# Autodesk Inventor assembly: assembly
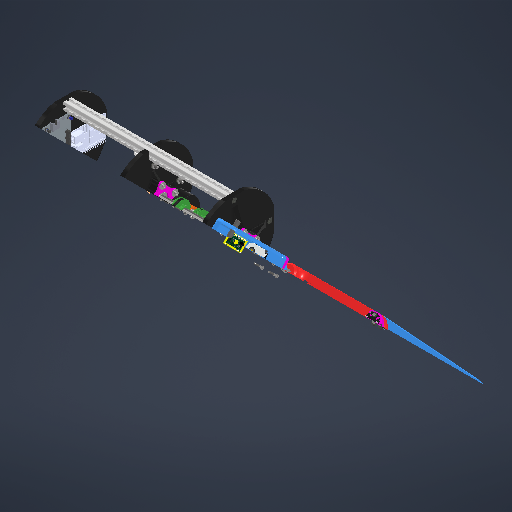
[picture p0: Inventor's stored thumbnail of the model, 512x512]
Saved by Autodesk Inventor 2027.1 (Build 311270010, 270A)
## iProperties
Created: 2026-10-07
Part Number: assembly
Document SubType Name: Assembly
Designer: luca
Author: luca
## Documents named in this file (71)
- C:\Users\lucao\Desktop\RL-Rotary-Inverted-Double-Pendulum\CAD\assembly.iam
- C:\Users\lucao\Desktop\RL-Rotary-Inverted-Double-Pendulum\CAD\motor\L-7015-251029\2D3D\RMD-7015三维图\RMD-7015\RMD-7015.ipt
- C:\Users\lucao\Desktop\RL-Rotary-Inverted-Double-Pendulum\CAD\encoder\AMT102-D2048-I6350-S\3D\AMT102-D2048-I6350-S\AMT102-D2048-I6350-S.ipt
- C:\Users\lucao\Desktop\RL-Rotary-Inverted-Double-Pendulum\CAD\Electronics\RASPBERRY_PI_5\RASPBERRY_PI_5.ipt
- C:\Users\lucao\Desktop\RL-Rotary-Inverted-Double-Pendulum\CAD\Electronics\stm32\NUCLEO-F429ZI--3DModel-STEP-56544\NUCLEO-F429ZI--3DModel-STEP-56544.ipt
- C:\Users\lucao\Desktop\RL-Rotary-Inverted-Double-Pendulum\CAD\al-profil-20x20-drazka-6\al-profil-20x20-drazka-6.ipt
- C:\Users\lucao\Desktop\RL-Rotary-Inverted-Double-Pendulum\CAD\plate_lower.ipt
- C:\Users\lucao\Desktop\RL-Rotary-Inverted-Double-Pendulum\CAD\plate_middle.ipt
- C:\Users\lucao\Desktop\RL-Rotary-Inverted-Double-Pendulum\CAD\drive_shaft_center.ipt
- C:\Users\lucao\Desktop\RL-Rotary-Inverted-Double-Pendulum\CAD\plate_upper.ipt
- C:\Users\lucao\Desktop\RL-Rotary-Inverted-Double-Pendulum\CAD\motor_driveshaft.ipt
- C:\Users\lucao\Desktop\RL-Rotary-Inverted-Double-Pendulum\CAD\90_Deg_Profile\90_Deg_Profile.ipt
- C:\Users\lucao\Desktop\RL-Rotary-Inverted-Double-Pendulum\CAD\pulleyGT3_12mm.ipt
- C:\Users\lucao\Desktop\RL-Rotary-Inverted-Double-Pendulum\CAD\pulleyGT3_17mm.ipt
- C:\Users\lucao\Documents\Inventor\Content Center Files\R2027\en-US\DIN 625 - T1\DIN 625 T1 - 16003 - 17 x 35 x 8.ipt
- C:\Users\lucao\Desktop\RL-Rotary-Inverted-Double-Pendulum\CAD\motor_flange.ipt
- C:\Users\lucao\Documents\Inventor\Content Center Files\R2027\en-US\DIN EN ISO 7091\DIN EN ISO 7091 - 4.ipt
- C:\Users\lucao\Documents\Inventor\Content Center Files\R2027\en-US\ISO 4762(1)\DIN EN ISO 4762 - M4 x 20.ipt
- C:\Users\lucao\Documents\Inventor\Content Center Files\R2027\en-US\ISO 4032(1)\ISO 4032 - M4DIN EN.ipt
- C:\Users\lucao\Documents\Inventor\Content Center Files\R2027\en-US\DIN 914\DIN 914 - M4 x 12.ipt
- C:\Users\lucao\Desktop\RL-Rotary-Inverted-Double-Pendulum\CAD\bearing_lock_middleplate_upper.ipt
- C:\Users\lucao\Desktop\RL-Rotary-Inverted-Double-Pendulum\CAD\bearing_distancer_middle.ipt
- C:\Users\lucao\Documents\Inventor\Content Center Files\R2027\en-US\DIN 9021\DIN 9021 - 5,3.ipt
- C:\Users\lucao\Documents\Inventor\Content Center Files\R2027\en-US\ISO 4762(1)\DIN EN ISO 4762 - M5 x 40.ipt
- C:\Users\lucao\Documents\Inventor\Content Center Files\R2027\en-US\ISO 4032(1)\ISO 4032 - M5DIN EN.ipt
- C:\Users\lucao\Documents\Inventor\Content Center Files\R2027\en-US\ISO 4762(1)\DIN EN ISO 4762 - M3 x 16.ipt
- C:\Users\lucao\Documents\Inventor\Content Center Files\R2027\en-US\DIN EN ISO 7091\DIN EN ISO 7091 - 3.ipt
- C:\Users\lucao\Desktop\RL-Rotary-Inverted-Double-Pendulum\CAD\timing_belt.ipt
- C:\Users\lucao\Documents\Inventor\Content Center Files\R2027\en-US\ISO 10642(2)\ISO 10642  - M6  x  45.ipt
- C:\Users\lucao\Documents\Inventor\Content Center Files\R2027\en-US\ISO 4762(1)\DIN EN ISO 4762 - M6 x 25.ipt
- C:\Users\lucao\Documents\Inventor\Content Center Files\R2027\en-US\ISO 7091\ISO 7091 - ST 6 - 100 HV.ipt
- C:\Users\lucao\Documents\Inventor\Content Center Files\R2027\en-US\ISO 4036(1)\ISO 4036 - M6(1).ipt
- C:\Users\lucao\Desktop\RL-Rotary-Inverted-Double-Pendulum\CAD\axialLock_mainShaft.ipt
- C:\Users\lucao\Documents\Inventor\Content Center Files\R2027\en-US\DIN 914\DIN 914 - M3 x 6.ipt
- C:\Users\lucao\Documents\Inventor\Content Center Files\R2027\en-US\DIN EN ISO 4036\DIN EN ISO 4036 - M3.ipt
- C:\Users\lucao\Desktop\RL-Rotary-Inverted-Double-Pendulum\CAD\link_mainaxis_to_horArm.ipt
- C:\Users\lucao\Documents\Inventor\Content Center Files\R2027\en-US\DIN BEARING(1)\DIN 625 SKF - SKF 6001.ipt
- C:\Users\lucao\Desktop\RL-Rotary-Inverted-Double-Pendulum\CAD\drive_shaft_arm.ipt
- C:\Users\lucao\Desktop\RL-Rotary-Inverted-Double-Pendulum\CAD\slipringMountArm.ipt
- C:\Users\lucao\Desktop\RL-Rotary-Inverted-Double-Pendulum\CAD\slipRing.ipt
- C:\Users\lucao\Desktop\RL-Rotary-Inverted-Double-Pendulum\CAD\distanceTube_armshaft.ipt
- C:\Users\lucao\Desktop\RL-Rotary-Inverted-Double-Pendulum\CAD\slipRingMount_mainAxis.ipt
- C:\Users\lucao\Desktop\RL-Rotary-Inverted-Double-Pendulum\CAD\plate_arm_bearing_fix.ipt
- C:\Users\lucao\Documents\Inventor\Content Center Files\R2027\en-US\DIN 6912\DIN 6912 - M4 x 25.ipt
- C:\Users\lucao\Desktop\RL-Rotary-Inverted-Double-Pendulum\CAD\slipring_tube.ipt
- C:\Users\lucao\Desktop\RL-Rotary-Inverted-Double-Pendulum\CAD\Insert M3 D5 L5mm\Insert M3 D5 L5mm.ipt
- C:\Users\lucao\Documents\Inventor\Content Center Files\R2027\en-US\CNS 4481\CNS 4481 - M3 x 5.ipt
- C:\Users\lucao\Documents\Inventor\Content Center Files\R2027\en-US\CNS 4481\CNS 4481 - M3 x 6.ipt
- C:\Users\lucao\Documents\Inventor\Content Center Files\R2027\en-US\DIN 7984\DIN 7984 - M3 x 6.ipt
- C:\Users\lucao\Desktop\RL-Rotary-Inverted-Double-Pendulum\CAD\STM32 Mini F401\STM32MiniF401.iam
- C:\Users\lucao\Desktop\RL-Rotary-Inverted-Double-Pendulum\CAD\weight_rod.ipt
- C:\Users\lucao\Desktop\RL-Rotary-Inverted-Double-Pendulum\CAD\axialLock_arm.ipt
- C:\Users\lucao\Documents\Inventor\Content Center Files\R2027\en-US\DIN 914\DIN 914 - M3 x 8.ipt
- C:\Users\lucao\Desktop\RL-Rotary-Inverted-Double-Pendulum\CAD\pendulum_1.ipt
- C:\Users\lucao\Documents\Inventor\Content Center Files\R2027\en-US\DIN BEARING(1)\DIN 625 SKF - SKF 608.ipt
- C:\Users\lucao\Desktop\RL-Rotary-Inverted-Double-Pendulum\CAD\pendulum_2.ipt
- C:\Users\lucao\Desktop\RL-Rotary-Inverted-Double-Pendulum\CAD\rod_link1to2.ipt
- C:\Users\lucao\Documents\Inventor\Content Center Files\R2027\en-US\DIN 7349\DIN 7349 - 4,3.ipt
- C:\Users\lucao\Documents\Inventor\Content Center Files\R2027\en-US\CSN EN 24017\ISO 4017 - M4 x 8CSN EN.ipt
- C:\Users\lucao\Desktop\RL-Rotary-Inverted-Double-Pendulum\CAD\sensormout_pendulum.ipt
- C:\Users\lucao\Desktop\RL-Rotary-Inverted-Double-Pendulum\CAD\mt6701.ipt
- C:\Users\lucao\Desktop\RL-Rotary-Inverted-Double-Pendulum\CAD\magnet.ipt
- C:\Users\lucao\Desktop\RL-Rotary-Inverted-Double-Pendulum\CAD\Insert M3 D5 L5mm\Insert M3 D5 L5mm_MIR.ipt
- C:\Users\lucao\Documents\Inventor\Content Center Files\R2027\en-US\DIN 7349\DIN 7349 - 3,2.ipt
- C:\Users\lucao\Documents\Inventor\Content Center Files\R2027\en-US\ISO 4762(1)\DIN EN ISO 4762 - M3 x 8.ipt
- C:\Users\lucao\Documents\Inventor\Content Center Files\R2027\en-US\ISO 10642(2)\ISO 10642  - M3  x  16.ipt
- C:\Users\lucao\Documents\Inventor\Content Center Files\R2027\en-US\DIN EN 24 036(2)\DIN EN 24 036 - M3.ipt
- C:\Users\lucao\Desktop\RL-Rotary-Inverted-Double-Pendulum\CAD\Insert M3 D5 L5mm\Insert M3 D5 L5mm_MIR1.ipt
- C:\Users\lucao\Documents\Inventor\Content Center Files\R2027\en-US\ISO 10642(2)\ISO 10642  - M3  x  10.ipt
- C:\Users\lucao\Documents\Inventor\Content Center Files\R2027\en-US\DIN EN ISO 4027\DIN EN ISO 4027 - M3 x 16.ipt
- C:\Users\lucao\Desktop\RL-Rotary-Inverted-Double-Pendulum\CAD\Insert M3 D5 L5mm\Insert M3 D5 L5mm_MIR2.ipt
## Components (197 placed, 70 different names)
1. RASPBERRY_PI_5:1 — Mate:7
2. NUCLEO-F429ZI--3DModel-STEP-56544:1 — Mate:6
3. timing_belt:1 — Mate:91, Mate:92, Mate:93
4. RMD-7015:1 — Mate:11, Mate:34, Mate:35, Angle:4, Mate:57, Mate:58, Mate:72, Mate:74, Mate:75, Mate:76, Mate:77, Mate:78
5. motor_driveshaft:1 — Mate:34, Mate:35, Mate:55, Mate:56, Mate:91
6. pulleyGT3_12mm:1 — Mate:55, Mate:71, Flush:5, Mate:93
7. motor_flange:1 — Mate:56, Mate:57, Insert:1, Insert:2, Insert:3, Insert:4, Insert:9, Mate:58, Flush:4, Mate:71
8. DIN EN ISO 7091 4:1 — Insert:1, Insert:5
9. DIN EN ISO 7091 4:2 — Insert:2, Insert:8
10. DIN EN ISO 7091 4:3 — Insert:3, Insert:7
11. DIN EN ISO 7091 4:4 — Insert:4, Insert:6
12. DIN EN ISO 4762 M4 x 20:1 — Insert:5
13. DIN EN ISO 4762 M4 x 20:2 — Insert:6
14. DIN EN ISO 4762 M4 x 20:3 — Insert:7
15. DIN EN ISO 4762 M4 x 20:4 — Insert:8
16. DIN 625 - T1 16003 - 17 x 35 x 8:4 — Mate:53, Mate:132, Mate:133, Mate:136
17. DIN 625 - T1 16003 - 17 x 35 x 8:3 — Mate:52, Mate:129, Mate:131, Mate:149
18. DIN 625 - T1 16003 - 17 x 35 x 8:2 — Mate:51, Mate:63, Mate:69
19. DIN 625 - T1 16003 - 17 x 35 x 8:1 — Mate:50, Mate:65, Mate:67, Mate:70, Flush:6
20. DIN EN 24032 M5:4 — Insert:22
21. DIN EN 24032 M5:3 — Insert:21
22. DIN EN 24032 M5:2 — Insert:20
23. DIN EN 24032 M5:1 — Insert:19
24. DIN EN ISO 7091 3:4 — Mate:85, Mate:86, Mate:90
25. DIN EN ISO 7091 3:3 — Mate:83, Mate:84, Mate:89
26. DIN EN ISO 7091 3:2 — Mate:81, Mate:82, Mate:87
27. DIN EN ISO 7091 3:1 — Mate:79, Mate:80, Mate:88
28. DIN EN ISO 4762 M3 x 16:4 — Mate:77, Mate:79, Mate:88
29. DIN EN ISO 4762 M3 x 16:3 — Mate:76, Mate:83, Mate:89
30. DIN EN ISO 4762 M3 x 16:2 — Mate:78, Mate:85, Mate:90
31. DIN EN ISO 4762 M3 x 16:1 — Mate:75, Mate:81, Mate:87
32. bearing_distancer_middle:2 — Mate:130, Mate:131, Mate:132
33. bearing_distancer_middle:1 — Mate:68, Mate:69, Mate:70
34. plate_lower:1 — Mate:1, Mate:2, Mate:3, Mate:4, Mate:5, Angle:1, Mate:6, Mate:7, Mate:17, Mate:19, Mate:98, Mate:99, Mate:100, Mate:101
35. DIN EN ISO 10642 M6  x  45:4 — Mate:97
36. DIN EN ISO 10642 M6  x  45:2 — Mate:95
37. DIN EN ISO 10642 M6  x  45:1 — Mate:94
38. DIN EN ISO 10642 M6  x  45:3 — Mate:96
39. DIN EN ISO 10642 M6  x  45:6 — Mate:99
40. DIN EN ISO 10642 M6  x  45:7 — Mate:100
41. DIN EN ISO 10642 M6  x  45:5 — Mate:98
42. DIN EN ISO 10642 M6  x  45:8 — Mate:101
43. plate_middle:1 — Mate:11, Mate:17, Mate:19, Angle:2, Mate:42, Mate:62, Mate:66, Mate:67, Insert:14, Mate:80, Mate:82, Mate:84, Mate:86, Mate:102, Mate:104, Mate:106, Mate:108, Mate:111, Mate:113, Mate:115, Mate:117
44. plate_upper:1 — Mate:18, Mate:20, Mate:21, Angle:3, Mate:94, Mate:95, Mate:96, Mate:97, Mate:133, Mate:134, Mate:142
45. bearing_lock_middleplate_upper:1 — Mate:61, Mate:62, Mate:63, Insert:10, Insert:11, Insert:12, Insert:13
46. DIN 9021 5,3:1 — Insert:10, Insert:18
47. DIN 9021 5,3:2 — Insert:11, Insert:17
48. DIN 9021 5,3:3 — Insert:12, Insert:15
49. DIN 9021 5,3:4 — Insert:13, Insert:16
50. DIN EN ISO 4762 M5 x 40:1 — Insert:15
51. DIN EN ISO 4762 M5 x 40:2 — Insert:16
52. DIN EN ISO 4762 M5 x 40:3 — Insert:17
53. DIN EN ISO 4762 M5 x 40:4 — Insert:18
54. DIN EN ISO 4762 M6 x 25:1 — Mate:102, Mate:103, Mate:110, Mate:120
55. DIN EN ISO 4762 M6 x 25:2 — Mate:104, Mate:105, Mate:116, Mate:118
56. DIN EN ISO 4762 M6 x 25:3 — Mate:106, Mate:107, Mate:114, Mate:122
57. DIN EN ISO 4762 M6 x 25:4 — Mate:108, Mate:109, Mate:112, Mate:124
58. ISO 7091 ST 6 - 100 HV:1 — Mate:110, Mate:111, Mate:121
59. ISO 7091 ST 6 - 100 HV:2 — Mate:112, Mate:113, Mate:125
60. ISO 7091 ST 6 - 100 HV:3 — Mate:114, Mate:115, Mate:123
61. ISO 7091 ST 6 - 100 HV:4 — Mate:116, Mate:117, Mate:119
62. DIN EN 24036 M6:1 — Mate:118, Mate:119
63. DIN EN 24036 M6:2 — Mate:120, Mate:121
64. DIN EN 24036 M6:3 — Mate:122, Mate:123
65. DIN EN 24036 M6:4 — Mate:124, Mate:125
66. bearing_lock_middleplate_upper:2 — Mate:128, Mate:129, Mate:134, Mate:137, Mate:139
67. axialLock_arm:1 — Mate:194, Mate:195, Mate:196, Angle:9, Mate:197, Mate:198, Mate:199
68. slipRing:1 — Mate:178, Flush:9
69. slipring_tube:1 — Mate:176, Mate:177, Mate:178, Flush:9, Flush:13
70. slipringMountArm:1 — Mate:174, Mate:175, Mate:179, Flush:10, Mate:180, Flush:11, Mate:181, Mate:182, Mate:183, Flush:12
71. drive_shaft_arm:1 — Mate:154, Mate:158, Mate:165, Flush:8, Mate:174, Mate:176, Mate:194, Mate:202, Flush:17
72. pendulum_1:1 — Mate:202, Flush:17, Mate:203, Mate:217, Mate:219, Mate:223, Mate:234, Angle:11, Mate:235, Flush:20, Mate:240, Mate:241, Angle:12, Flush:22, Flush:23, Mate:249, Flush:29
73. DIN 625 SKF SKF 608:1 — Mate:203, Mate:206, Mate:208, Mate:211, Mate:220, Mate:223
74. sensormout_pendulum:1 — Mate:217, Mate:219, Mate:220, Mate:222, Mate:229, Flush:19, Mate:232, Mate:236, Mate:237, Flush:21, Mate:248
75. mt6701:1 — Mate:221, Mate:222, Mate:226, Mate:230, Mate:231, Mate:239
76. Insert M3 D5 L5mm:11 — Mate:229, Flush:19
77. Insert M3 D5 L5mm_MIR:1 — Flush:21, Mate:238
78. DIN 7349 3,2:1 — Mate:230, Mate:231, Insert:34
79. DIN EN ISO 4762 M3 x 8:1 — Insert:34
80. DIN 7349 3,2:2 — Insert:35, Mate:239
81. DIN EN ISO 4762 M3 x 8:2 — Insert:35, Mate:238, Mate:248
82. DIN EN ISO 10642 M3  x  16:1 — Mate:232, Mate:233
83. DIN EN 24036 M3:1 — Mate:233, Mate:234, Angle:11
84. Insert M3 D5 L5mm:12 — Mate:235, Flush:20
85. Insert M3 D5 L5mm_MIR1:1 — Mate:249, Flush:29
86. DIN EN ISO 10642 M3  x  10:1 — Mate:236
87. DIN EN ISO 10642 M3  x  10:2 — Mate:237
88. DIN EN 24032 M4:9 — Mate:240, Mate:241, Angle:12, Mate:242
89. DIN 914 M4 x 12:5 — Mate:242, Flush:22
90. AMT102-D2048-I6350-S:1 — Mate:173, Angle:7, Mate:177, Flush:13, Mate:187, Mate:189
91. pulleyGT3_17mm:1 — Mate:54, Flush:5
92. drive_shaft_center:1 — Mate:50, Mate:51, Mate:52, Mate:53, Mate:54, Mate:61, Mate:66, Mate:68, Mate:72, Mate:92, Mate:128, Mate:130, Mate:135, Flush:6, Flush:7, Mate:148, Mate:161, Mate:162, Angle:8
93. DIN 625 SKF SKF 6001:2 — Mate:151, Mate:160, Mate:164, Mate:175
94. DIN 625 SKF SKF 6001:3 — Mate:154, Mate:159, Mate:163, Mate:190, Mate:195
95. distanceTube_armshaft:1 — Mate:158, Mate:159, Mate:160
96. slipRingMount_mainAxis:1 — Mate:161, Mate:162, Mate:243, Flush:24
97. plate_arm_bearing_fix:1 — Mate:165, Mate:166, Insert:25, Insert:26, Insert:27, Insert:28, Mate:190
98. DIN EN ISO 7091 4:7 — Insert:25, Insert:29
99. DIN EN ISO 7091 4:8 — Insert:26, Insert:30
100. DIN EN ISO 7091 4:9 — Insert:27, Insert:31
101. DIN EN ISO 7091 4:10 — Insert:28, Insert:32
102. DIN 6912 M4 x 25:1 — Insert:29, Mate:200
103. DIN 6912 M4 x 25:2 — Insert:30
104. DIN 6912 M4 x 25:3 — Insert:31
105. DIN 6912 M4 x 25:4 — Insert:32
106. Insert M3 D5 L5mm:9 — Mate:184, Flush:14
107. Insert M3 D5 L5mm:10 — Mate:185, Flush:15
108. DIN 7984 M3 x 6:1 — Mate:186, Mate:187
109. DIN 7984 M3 x 6:2 — Mate:188, Mate:189
110. STM32MiniF401:1 [sub-assembly] — Mate:191, Mate:192
111. weight_rod:1 — Mate:193, Flush:16
112. DIN EN 24032 M4:5 — Mate:200, Mate:201, Angle:10
113. DIN EN 24032 M4:6
114. DIN EN 24032 M4:7
115. DIN EN 24032 M4:8
116. slipRing:2 — Mate:243, Flush:24
117. Insert M3 D5 L5mm:13 — Mate:244, Flush:25, Mate:245
118. DIN EN ISO 4027 M3 x 16:1 — Mate:245, Flush:28
119. Insert M3 D5 L5mm_MIR2:1 — Mate:246, Mate:247, Flush:26
120. DIN EN ISO 4027 M3 x 16:2 — Mate:246, Flush:27
121. axialLock_mainShaft:1 — Mate:135, Mate:136, Mate:145, Angle:6, Mate:147
122. link_mainaxis_to_horArm:1 — Mate:148, Mate:149, Mate:151, Mate:152, Mate:163, Mate:164, Mate:166, Mate:173, Angle:7, Flush:8, Mate:184, Flush:14, Mate:185, Flush:15, Mate:186, Mate:188, Angle:8, Mate:191, Mate:192, Mate:193, Flush:16, Mate:201, Angle:10, Mate:244, Flush:25, Mate:247, Flush:26, Flush:27, Flush:28
123. magnet:1 — Mate:224, Mate:225, Mate:226
124. pendulum_2:1 — Mate:206, Mate:208, Mate:209, Flush:18, Mate:213
125. rod_link1to2:1 — Mate:209, Flush:18, Mate:210, Mate:212, Mate:214
126. DIN 7349 4,3:1 — Mate:210, Mate:211, Insert:33, Mate:221, Mate:225
127. DIN 7349 4,3:2 — Mate:212, Mate:213, Mate:215
128. CSN EN 24017 M4 x 8:1 — Insert:33, Mate:224
129. CSN EN 24017 M4 x 8:2 — Mate:214, Mate:215
130. DIN EN 24032 M4:1 — Insert:9, Mate:59
131. DIN EN 24032 M4:2
132. DIN EN 24032 M4:3
133. DIN EN 24032 M4:4
134. DIN 914 M4 x 12:1 — Mate:59, Flush:4
135. DIN 914 M4 x 12:2
136. DIN 914 M4 x 12:3
137. DIN 914 M4 x 12:4
138. DIN 9021 5,3:5 — Insert:14, Insert:22
139. DIN 9021 5,3:6 — Insert:21
140. DIN 9021 5,3:7 — Insert:20
141. DIN 9021 5,3:8 — Insert:19
142. al-profil-20x20-drazka-6:1 — Mate:4, Mate:5, Angle:1, Mate:20, Mate:21
143. al-profil-20x20-drazka-6:2 — Mate:18, Angle:2, Angle:3
144. al-profil-20x20-drazka-6:3
145. al-profil-20x20-drazka-6:4 — Flush:1, Mate:43
146. 90_Deg_Profile:1 — Mate:42, Flush:1, Mate:43, Mate:103, Mate:105, Mate:107, Mate:109
147. 90_Deg_Profile:2
148. 90_Deg_Profile:3
149. 90_Deg_Profile:4
150. DIN EN 24032 M5:5 — Mate:143, Mate:144
151. DIN EN ISO 4762 M5 x 40:5 — Mate:137, Mate:138, Mate:140, Mate:141, Mate:144
152. DIN 9021 5,3:10 — Mate:141, Mate:142, Mate:143
153. DIN 9021 5,3:9 — Mate:138, Mate:139, Mate:140
154. DIN EN 24032 M5:6
155. DIN EN ISO 4762 M5 x 40:6
156. DIN 9021 5,3:11
157. DIN 9021 5,3:12
158. DIN EN 24032 M5:7
159. DIN EN ISO 4762 M5 x 40:7
160. DIN 9021 5,3:13
161. DIN 9021 5,3:14
162. DIN EN 24032 M5:8
163. DIN EN ISO 4762 M5 x 40:8
164. DIN 9021 5,3:15
165. DIN 9021 5,3:16
166. DIN 914 M3 x 8:1 — Mate:198, Mate:199
167. DIN 914 M3 x 8:2
168. DIN 914 M3 x 8:3
169. DIN 914 M3 x 8:4
170. DIN EN ISO 4036 M3:5 — Mate:196, Angle:9, Mate:197
171. DIN EN ISO 4036 M3:6
172. DIN EN ISO 4036 M3:7
173. DIN EN ISO 4036 M3:8
174. Insert M3 D5 L5mm:1 — Mate:179, Flush:10
175. Insert M3 D5 L5mm:2
176. Insert M3 D5 L5mm:3
177. Insert M3 D5 L5mm:4
178. Insert M3 D5 L5mm:5 — Mate:180, Flush:11
179. Insert M3 D5 L5mm:6
180. Insert M3 D5 L5mm:7
181. Insert M3 D5 L5mm:8
182. CNS 4481 M3 x 5:1 — Mate:181, Mate:182
183. CNS 4481 M3 x 5:2
184. CNS 4481 M3 x 5:3
185. CNS 4481 M3 x 5:4
186. CNS 4481 M3 x 6:3 — Mate:183, Flush:12
187. CNS 4481 M3 x 6:4
188. CNS 4481 M3 x 6:5
189. CNS 4481 M3 x 6:6
190. DIN 914 M3 x 6:1 — Mate:145, Flush:7
191. DIN 914 M3 x 6:2 — Mate:146
192. DIN 914 M3 x 6:3
193. DIN 914 M3 x 6:4
194. DIN EN ISO 4036 M3:1 — Mate:146, Angle:6, Mate:147
195. DIN EN ISO 4036 M3:2
196. DIN EN ISO 4036 M3:3
197. DIN EN ISO 4036 M3:4
## Component patterns: (4 elements, first: DIN EN 24032 M4:1), (4 elements, first: DIN 914 M4 x 12:1), (4 elements, first: DIN 9021 5,3:5), (4 elements, first: al-profil-20x20-drazka-6:1), (4 elements, first: 90_Deg_Profile:1), (4 elements, first: DIN EN 24032 M5:5 + DIN EN ISO 4762 M5 x 40:5 + DIN 9021 5,3:10 + DIN 9021 5,3:9), (4 elements, first: DIN 914 M3 x 8:1), (4 elements, first: DIN EN ISO 4036 M3:5), (4 elements, first: Insert M3 D5 L5mm:1), (4 elements, first: Insert M3 D5 L5mm:5), (4 elements, first: CNS 4481 M3 x 5:1), (4 elements, first: CNS 4481 M3 x 6:3), (4 elements, first: DIN 914 M3 x 6:1), (4 elements, first: DIN EN ISO 4036 M3:1)
## Relationships (267: Mate 195, Insert 33, Flush 27, Angle 12)
- Mate:1: plate_lower:1
- Mate:2: plate_lower:1
- Mate:3: plate_lower:1
- Mate:4: plate_lower:1 ↔ al-profil-20x20-drazka-6:1
- Mate:5: plate_lower:1 ↔ al-profil-20x20-drazka-6:1
- Angle:1 (0 deg): plate_lower:1 ↔ al-profil-20x20-drazka-6:1
- Mate:6: NUCLEO-F429ZI--3DModel-STEP-56544:1 ↔ plate_lower:1
- Mate:7: RASPBERRY_PI_5:1 ↔ plate_lower:1
- Mate:11: RMD-7015:1 ↔ plate_middle:1
- Mate:17 (200 mm): plate_lower:1 ↔ plate_middle:1
- Mate:18: plate_upper:1 ↔ al-profil-20x20-drazka-6:2
- Mate:19: plate_lower:1 ↔ plate_middle:1
- Angle:2 (0 deg): plate_middle:1 ↔ al-profil-20x20-drazka-6:2
- Mate:20: plate_upper:1 ↔ al-profil-20x20-drazka-6:1
- Mate:21: plate_upper:1 ↔ al-profil-20x20-drazka-6:1
- Angle:3 (0 deg): plate_upper:1 ↔ al-profil-20x20-drazka-6:2
- Mate:34: RMD-7015:1 ↔ motor_driveshaft:1
- Mate:35: RMD-7015:1 ↔ motor_driveshaft:1
- Mate:42: plate_middle:1 ↔ 90_Deg_Profile:1
- Flush:1: al-profil-20x20-drazka-6:4 ↔ 90_Deg_Profile:1
- Mate:43: al-profil-20x20-drazka-6:4 ↔ 90_Deg_Profile:1
- Angle:4 (0 deg): RMD-7015:1
- Mate:50: DIN 625 - T1 16003 - 17 x 35 x 8:1 ↔ drive_shaft_center:1
- Mate:51: DIN 625 - T1 16003 - 17 x 35 x 8:2 ↔ drive_shaft_center:1
- Mate:52: DIN 625 - T1 16003 - 17 x 35 x 8:3 ↔ drive_shaft_center:1
- Mate:53: DIN 625 - T1 16003 - 17 x 35 x 8:4 ↔ drive_shaft_center:1
- Mate:54: pulleyGT3_17mm:1 ↔ drive_shaft_center:1
- Mate:55: motor_driveshaft:1 ↔ pulleyGT3_12mm:1
- Mate:56: motor_driveshaft:1 ↔ motor_flange:1
- Mate:57: RMD-7015:1 ↔ motor_flange:1
- Insert:1: motor_flange:1 ↔ DIN EN ISO 7091 4:1
- Insert:2: motor_flange:1 ↔ DIN EN ISO 7091 4:2
- Insert:3: motor_flange:1 ↔ DIN EN ISO 7091 4:3
- Insert:4: motor_flange:1 ↔ DIN EN ISO 7091 4:4
- Insert:5: DIN EN ISO 7091 4:1 ↔ DIN EN ISO 4762 M4 x 20:1
- Insert:6: DIN EN ISO 7091 4:4 ↔ DIN EN ISO 4762 M4 x 20:2
- Insert:7: DIN EN ISO 7091 4:3 ↔ DIN EN ISO 4762 M4 x 20:3
- Insert:8: DIN EN ISO 7091 4:2 ↔ DIN EN ISO 4762 M4 x 20:4
- Insert:9: motor_flange:1 ↔ DIN EN 24032 M4:1
- Mate:58: RMD-7015:1 ↔ motor_flange:1
- Mate:59: DIN EN 24032 M4:1 ↔ DIN 914 M4 x 12:1
- Flush:4: motor_flange:1 ↔ DIN 914 M4 x 12:1
- Mate:61: bearing_lock_middleplate_upper:1 ↔ drive_shaft_center:1
- Mate:62: plate_middle:1 ↔ bearing_lock_middleplate_upper:1
- Mate:63: DIN 625 - T1 16003 - 17 x 35 x 8:2 ↔ bearing_lock_middleplate_upper:1
- Mate:65: DIN 625 - T1 16003 - 17 x 35 x 8:1
- Mate:66: plate_middle:1 ↔ drive_shaft_center:1
- Mate:67: DIN 625 - T1 16003 - 17 x 35 x 8:1 ↔ plate_middle:1
- Mate:68: bearing_distancer_middle:1 ↔ drive_shaft_center:1
- Mate:69: DIN 625 - T1 16003 - 17 x 35 x 8:2 ↔ bearing_distancer_middle:1
- Mate:70: DIN 625 - T1 16003 - 17 x 35 x 8:1 ↔ bearing_distancer_middle:1
- Insert:10: bearing_lock_middleplate_upper:1 ↔ DIN 9021 5,3:1
- Insert:11: bearing_lock_middleplate_upper:1 ↔ DIN 9021 5,3:2
- Insert:12: bearing_lock_middleplate_upper:1 ↔ DIN 9021 5,3:3
- Insert:13: bearing_lock_middleplate_upper:1 ↔ DIN 9021 5,3:4
- Insert:14: plate_middle:1 ↔ DIN 9021 5,3:5
- Insert:15: DIN 9021 5,3:3 ↔ DIN EN ISO 4762 M5 x 40:1
- Insert:16: DIN 9021 5,3:4 ↔ DIN EN ISO 4762 M5 x 40:2
- Insert:17: DIN 9021 5,3:2 ↔ DIN EN ISO 4762 M5 x 40:3
- Insert:18: DIN 9021 5,3:1 ↔ DIN EN ISO 4762 M5 x 40:4
- Insert:19: DIN EN 24032 M5:1 ↔ DIN 9021 5,3:8
- Insert:20: DIN EN 24032 M5:2 ↔ DIN 9021 5,3:7
- Insert:21: DIN EN 24032 M5:3 ↔ DIN 9021 5,3:6
- Insert:22: DIN EN 24032 M5:4 ↔ DIN 9021 5,3:5
- Mate:71 (10 mm): pulleyGT3_12mm:1 ↔ motor_flange:1
- Flush:5: pulleyGT3_12mm:1 ↔ pulleyGT3_17mm:1
- Mate:72 (65.801 mm): RMD-7015:1 ↔ drive_shaft_center:1
- Mate:73
- Angle:5 (-45 deg)
- Mate:74: RMD-7015:1
- Mate:75: RMD-7015:1 ↔ DIN EN ISO 4762 M3 x 16:1
- Mate:76: RMD-7015:1 ↔ DIN EN ISO 4762 M3 x 16:3
- Mate:77: RMD-7015:1 ↔ DIN EN ISO 4762 M3 x 16:4
- Mate:78: RMD-7015:1 ↔ DIN EN ISO 4762 M3 x 16:2
- Mate:79: DIN EN ISO 7091 3:1 ↔ DIN EN ISO 4762 M3 x 16:4
- Mate:80: DIN EN ISO 7091 3:1 ↔ plate_middle:1
- Mate:81: DIN EN ISO 7091 3:2 ↔ DIN EN ISO 4762 M3 x 16:1
- Mate:82: DIN EN ISO 7091 3:2 ↔ plate_middle:1
- Mate:83: DIN EN ISO 7091 3:3 ↔ DIN EN ISO 4762 M3 x 16:3
- Mate:84: DIN EN ISO 7091 3:3 ↔ plate_middle:1
- Mate:85: DIN EN ISO 7091 3:4 ↔ DIN EN ISO 4762 M3 x 16:2
- Mate:86: DIN EN ISO 7091 3:4 ↔ plate_middle:1
- Mate:87: DIN EN ISO 7091 3:2 ↔ DIN EN ISO 4762 M3 x 16:1
- Mate:88: DIN EN ISO 7091 3:1 ↔ DIN EN ISO 4762 M3 x 16:4
- Mate:89: DIN EN ISO 7091 3:3 ↔ DIN EN ISO 4762 M3 x 16:3
- Mate:90: DIN EN ISO 7091 3:4 ↔ DIN EN ISO 4762 M3 x 16:2
- Mate:91: timing_belt:1 ↔ motor_driveshaft:1
- Mate:92: timing_belt:1 ↔ drive_shaft_center:1
- Mate:93 (1 mm): timing_belt:1 ↔ pulleyGT3_12mm:1
- Mate:94: DIN EN ISO 10642 M6  x  45:1 ↔ plate_upper:1
- Mate:95: DIN EN ISO 10642 M6  x  45:2 ↔ plate_upper:1
- Mate:96: DIN EN ISO 10642 M6  x  45:3 ↔ plate_upper:1
- Mate:97: DIN EN ISO 10642 M6  x  45:4 ↔ plate_upper:1
- Mate:98: plate_lower:1 ↔ DIN EN ISO 10642 M6  x  45:5
- Mate:99: plate_lower:1 ↔ DIN EN ISO 10642 M6  x  45:6
- Mate:100: plate_lower:1 ↔ DIN EN ISO 10642 M6  x  45:7
- Mate:101: plate_lower:1 ↔ DIN EN ISO 10642 M6  x  45:8
- Mate:102: plate_middle:1 ↔ DIN EN ISO 4762 M6 x 25:1
- Mate:103: DIN EN ISO 4762 M6 x 25:1 ↔ 90_Deg_Profile:1
- Mate:104: plate_middle:1 ↔ DIN EN ISO 4762 M6 x 25:2
- Mate:105: DIN EN ISO 4762 M6 x 25:2 ↔ 90_Deg_Profile:1
- Mate:106: plate_middle:1 ↔ DIN EN ISO 4762 M6 x 25:3
- Mate:107: DIN EN ISO 4762 M6 x 25:3 ↔ 90_Deg_Profile:1
- Mate:108: plate_middle:1 ↔ DIN EN ISO 4762 M6 x 25:4
- Mate:109: DIN EN ISO 4762 M6 x 25:4 ↔ 90_Deg_Profile:1
- Mate:110: DIN EN ISO 4762 M6 x 25:1 ↔ ISO 7091 ST 6 - 100 HV:1
- Mate:111: plate_middle:1 ↔ ISO 7091 ST 6 - 100 HV:1
- Mate:112: DIN EN ISO 4762 M6 x 25:4 ↔ ISO 7091 ST 6 - 100 HV:2
- Mate:113: plate_middle:1 ↔ ISO 7091 ST 6 - 100 HV:2
- Mate:114: DIN EN ISO 4762 M6 x 25:3 ↔ ISO 7091 ST 6 - 100 HV:3
- Mate:115: plate_middle:1 ↔ ISO 7091 ST 6 - 100 HV:3
- Mate:116: DIN EN ISO 4762 M6 x 25:2 ↔ ISO 7091 ST 6 - 100 HV:4
- Mate:117: plate_middle:1 ↔ ISO 7091 ST 6 - 100 HV:4
- Mate:118: DIN EN ISO 4762 M6 x 25:2 ↔ DIN EN 24036 M6:1
- Mate:119: ISO 7091 ST 6 - 100 HV:4 ↔ DIN EN 24036 M6:1
- Mate:120: DIN EN ISO 4762 M6 x 25:1 ↔ DIN EN 24036 M6:2
- Mate:121: ISO 7091 ST 6 - 100 HV:1 ↔ DIN EN 24036 M6:2
- Mate:122: DIN EN ISO 4762 M6 x 25:3 ↔ DIN EN 24036 M6:3
- Mate:123: ISO 7091 ST 6 - 100 HV:3 ↔ DIN EN 24036 M6:3
- Mate:124: DIN EN ISO 4762 M6 x 25:4 ↔ DIN EN 24036 M6:4
- Mate:125: ISO 7091 ST 6 - 100 HV:2 ↔ DIN EN 24036 M6:4
- Mate:128: bearing_lock_middleplate_upper:2 ↔ drive_shaft_center:1
- Mate:129: DIN 625 - T1 16003 - 17 x 35 x 8:3 ↔ bearing_lock_middleplate_upper:2
- Mate:130: bearing_distancer_middle:2 ↔ drive_shaft_center:1
- Mate:131: DIN 625 - T1 16003 - 17 x 35 x 8:3 ↔ bearing_distancer_middle:2
- Mate:132: DIN 625 - T1 16003 - 17 x 35 x 8:4 ↔ bearing_distancer_middle:2
- Mate:133: DIN 625 - T1 16003 - 17 x 35 x 8:4 ↔ plate_upper:1
- Mate:134: plate_upper:1 ↔ bearing_lock_middleplate_upper:2
- Mate:135: drive_shaft_center:1 ↔ axialLock_mainShaft:1
- Mate:136: DIN 625 - T1 16003 - 17 x 35 x 8:4 ↔ axialLock_mainShaft:1
- Flush:6 (-10 mm): DIN 625 - T1 16003 - 17 x 35 x 8:1 ↔ drive_shaft_center:1
- Mate:137: bearing_lock_middleplate_upper:2 ↔ DIN EN ISO 4762 M5 x 40:5
- Mate:138: DIN EN ISO 4762 M5 x 40:5 ↔ DIN 9021 5,3:9
- Mate:139: bearing_lock_middleplate_upper:2 ↔ DIN 9021 5,3:9
- Mate:140: DIN EN ISO 4762 M5 x 40:5 ↔ DIN 9021 5,3:9
- Mate:141: DIN EN ISO 4762 M5 x 40:5 ↔ DIN 9021 5,3:10
- Mate:142: plate_upper:1 ↔ DIN 9021 5,3:10
- Mate:143: DIN EN 24032 M5:5 ↔ DIN 9021 5,3:10
- Mate:144: DIN EN 24032 M5:5 ↔ DIN EN ISO 4762 M5 x 40:5
- Mate:145: axialLock_mainShaft:1 ↔ DIN 914 M3 x 6:1
- Flush:7 (-14.5 mm): drive_shaft_center:1 ↔ DIN 914 M3 x 6:1
- Mate:146: DIN 914 M3 x 6:2 ↔ DIN EN ISO 4036 M3:1
- Angle:6 (0 deg): axialLock_mainShaft:1 ↔ DIN EN ISO 4036 M3:1
- Mate:147: axialLock_mainShaft:1 ↔ DIN EN ISO 4036 M3:1
- Mate:148: drive_shaft_center:1 ↔ link_mainaxis_to_horArm:1
- Mate:149: DIN 625 - T1 16003 - 17 x 35 x 8:3 ↔ link_mainaxis_to_horArm:1
- Mate:151: DIN 625 SKF SKF 6001:2 ↔ link_mainaxis_to_horArm:1
- Mate:152: link_mainaxis_to_horArm:1
- Mate:154: drive_shaft_arm:1 ↔ DIN 625 SKF SKF 6001:3
- Mate:158: drive_shaft_arm:1 ↔ distanceTube_armshaft:1
- Mate:159: DIN 625 SKF SKF 6001:3 ↔ distanceTube_armshaft:1
- Mate:160: DIN 625 SKF SKF 6001:2 ↔ distanceTube_armshaft:1
- Mate:161: drive_shaft_center:1 ↔ slipRingMount_mainAxis:1
- Mate:162: drive_shaft_center:1 ↔ slipRingMount_mainAxis:1
- Mate:163: DIN 625 SKF SKF 6001:3 ↔ link_mainaxis_to_horArm:1
- Mate:164: DIN 625 SKF SKF 6001:2 ↔ link_mainaxis_to_horArm:1
- Mate:165: drive_shaft_arm:1 ↔ plate_arm_bearing_fix:1
- Mate:166: plate_arm_bearing_fix:1 ↔ link_mainaxis_to_horArm:1
- Insert:25: plate_arm_bearing_fix:1 ↔ DIN EN ISO 7091 4:7
- Insert:26: plate_arm_bearing_fix:1 ↔ DIN EN ISO 7091 4:8
- Insert:27: plate_arm_bearing_fix:1 ↔ DIN EN ISO 7091 4:9
- Insert:28: plate_arm_bearing_fix:1 ↔ DIN EN ISO 7091 4:10
- Insert:29: DIN EN ISO 7091 4:7 ↔ DIN 6912 M4 x 25:1
- Insert:30: DIN EN ISO 7091 4:8 ↔ DIN 6912 M4 x 25:2
- Insert:31: DIN EN ISO 7091 4:9 ↔ DIN 6912 M4 x 25:3
- Insert:32: DIN EN ISO 7091 4:10 ↔ DIN 6912 M4 x 25:4
- Mate:173: AMT102-D2048-I6350-S:1 ↔ link_mainaxis_to_horArm:1
- Angle:7 (180 deg): AMT102-D2048-I6350-S:1 ↔ link_mainaxis_to_horArm:1
- Flush:8 (5 mm): drive_shaft_arm:1 ↔ link_mainaxis_to_horArm:1
- Mate:174: slipringMountArm:1 ↔ drive_shaft_arm:1
- Mate:175: slipringMountArm:1 ↔ DIN 625 SKF SKF 6001:2
- Mate:176: slipring_tube:1 ↔ drive_shaft_arm:1
- Mate:177: slipring_tube:1 ↔ AMT102-D2048-I6350-S:1
- Mate:178: slipRing:1 ↔ slipring_tube:1
- Flush:9: slipRing:1 ↔ slipring_tube:1
- Mate:179: slipringMountArm:1 ↔ Insert M3 D5 L5mm:1
- Flush:10: slipringMountArm:1 ↔ Insert M3 D5 L5mm:1
- Mate:180: slipringMountArm:1 ↔ Insert M3 D5 L5mm:5
- Flush:11: slipringMountArm:1 ↔ Insert M3 D5 L5mm:5
- Mate:181: slipringMountArm:1 ↔ CNS 4481 M3 x 5:1
- Mate:182: slipringMountArm:1 ↔ CNS 4481 M3 x 5:1
- Mate:183: slipringMountArm:1 ↔ CNS 4481 M3 x 6:3
- Flush:12 (0.3 mm): slipringMountArm:1 ↔ CNS 4481 M3 x 6:3
- Flush:13: slipring_tube:1 ↔ AMT102-D2048-I6350-S:1
- Mate:184: Insert M3 D5 L5mm:9 ↔ link_mainaxis_to_horArm:1
- Flush:14: Insert M3 D5 L5mm:9 ↔ link_mainaxis_to_horArm:1
- Mate:185: Insert M3 D5 L5mm:10 ↔ link_mainaxis_to_horArm:1
- Flush:15: Insert M3 D5 L5mm:10 ↔ link_mainaxis_to_horArm:1
- Mate:186: DIN 7984 M3 x 6:1 ↔ link_mainaxis_to_horArm:1
- Mate:187: AMT102-D2048-I6350-S:1 ↔ DIN 7984 M3 x 6:1
- Mate:188: DIN 7984 M3 x 6:2 ↔ link_mainaxis_to_horArm:1
- Mate:189: AMT102-D2048-I6350-S:1 ↔ DIN 7984 M3 x 6:2
- Mate:190: DIN 625 SKF SKF 6001:3 ↔ plate_arm_bearing_fix:1
- Angle:8 (0 deg): drive_shaft_center:1 ↔ link_mainaxis_to_horArm:1
- Mate:191: STM32MiniF401:1 ↔ link_mainaxis_to_horArm:1
- Mate:192: STM32MiniF401:1 ↔ link_mainaxis_to_horArm:1
- Mate:193: weight_rod:1 ↔ link_mainaxis_to_horArm:1
- Flush:16 (-12.5 mm): weight_rod:1 ↔ link_mainaxis_to_horArm:1
- Mate:194: axialLock_arm:1 ↔ drive_shaft_arm:1
- Mate:195: axialLock_arm:1 ↔ DIN 625 SKF SKF 6001:3
- Mate:196: axialLock_arm:1 ↔ DIN EN ISO 4036 M3:5
- Angle:9 (0 deg): axialLock_arm:1 ↔ DIN EN ISO 4036 M3:5
- Mate:197: axialLock_arm:1 ↔ DIN EN ISO 4036 M3:5
- Mate:198: axialLock_arm:1 ↔ DIN 914 M3 x 8:1
- Mate:199 (-2 mm): axialLock_arm:1 ↔ DIN 914 M3 x 8:1
- Mate:200: DIN 6912 M4 x 25:1 ↔ DIN EN 24032 M4:5
- Mate:201: DIN EN 24032 M4:5 ↔ link_mainaxis_to_horArm:1
- Angle:10 (0 deg): DIN EN 24032 M4:5 ↔ link_mainaxis_to_horArm:1
- Mate:202: drive_shaft_arm:1 ↔ pendulum_1:1
- Flush:17: drive_shaft_arm:1 ↔ pendulum_1:1
- Mate:203: pendulum_1:1 ↔ DIN 625 SKF SKF 608:1
- Mate:206: DIN 625 SKF SKF 608:1 ↔ pendulum_2:1
- Mate:208: DIN 625 SKF SKF 608:1 ↔ pendulum_2:1
- Mate:209: pendulum_2:1 ↔ rod_link1to2:1
- Flush:18: pendulum_2:1 ↔ rod_link1to2:1
- Mate:210: rod_link1to2:1 ↔ DIN 7349 4,3:1
- Mate:211: DIN 625 SKF SKF 608:1 ↔ DIN 7349 4,3:1
- Mate:212: rod_link1to2:1 ↔ DIN 7349 4,3:2
- Mate:213: pendulum_2:1 ↔ DIN 7349 4,3:2
- Insert:33: DIN 7349 4,3:1 ↔ CSN EN 24017 M4 x 8:1
- Mate:214: rod_link1to2:1 ↔ CSN EN 24017 M4 x 8:2
- Mate:215: DIN 7349 4,3:2 ↔ CSN EN 24017 M4 x 8:2
- Mate:217: pendulum_1:1 ↔ sensormout_pendulum:1
- Mate:219: pendulum_1:1 ↔ sensormout_pendulum:1
- Mate:220: DIN 625 SKF SKF 608:1 ↔ sensormout_pendulum:1
- Mate:221: mt6701:1 ↔ DIN 7349 4,3:1
- Mate:222: sensormout_pendulum:1 ↔ mt6701:1
- Mate:223: pendulum_1:1 ↔ DIN 625 SKF SKF 608:1
- Mate:224: magnet:1 ↔ CSN EN 24017 M4 x 8:1
- Mate:225: magnet:1 ↔ DIN 7349 4,3:1
- Mate:226 (1.5 mm): mt6701:1 ↔ magnet:1
- Mate:229: sensormout_pendulum:1 ↔ Insert M3 D5 L5mm:11
- Flush:19: sensormout_pendulum:1 ↔ Insert M3 D5 L5mm:11
- Mate:230: mt6701:1 ↔ DIN 7349 3,2:1
- Mate:231: mt6701:1 ↔ DIN 7349 3,2:1
- Insert:34: DIN 7349 3,2:1 ↔ DIN EN ISO 4762 M3 x 8:1
- Insert:35: DIN 7349 3,2:2 ↔ DIN EN ISO 4762 M3 x 8:2
- Mate:232: sensormout_pendulum:1 ↔ DIN EN ISO 10642 M3  x  16:1
- Mate:233: DIN EN ISO 10642 M3  x  16:1 ↔ DIN EN 24036 M3:1
- Mate:234: pendulum_1:1 ↔ DIN EN 24036 M3:1
- Angle:11 (0 deg): pendulum_1:1 ↔ DIN EN 24036 M3:1
- Mate:235: pendulum_1:1 ↔ Insert M3 D5 L5mm:12
- Flush:20: pendulum_1:1 ↔ Insert M3 D5 L5mm:12
- Mate:236: sensormout_pendulum:1 ↔ DIN EN ISO 10642 M3  x  10:1
- Mate:237: sensormout_pendulum:1 ↔ DIN EN ISO 10642 M3  x  10:2
- Flush:21: sensormout_pendulum:1 ↔ Insert M3 D5 L5mm_MIR:1
- Mate:238: Insert M3 D5 L5mm_MIR:1 ↔ DIN EN ISO 4762 M3 x 8:2
- Mate:239: mt6701:1 ↔ DIN 7349 3,2:2
- Mate:240: pendulum_1:1 ↔ DIN EN 24032 M4:9
- Mate:241: pendulum_1:1 ↔ DIN EN 24032 M4:9
- Angle:12 (0 deg): pendulum_1:1 ↔ DIN EN 24032 M4:9
- Mate:242: DIN EN 24032 M4:9 ↔ DIN 914 M4 x 12:5
- Flush:22 (1 mm): pendulum_1:1 ↔ DIN 914 M4 x 12:5
- Flush:23: pendulum_1:1
- Mate:243: slipRingMount_mainAxis:1 ↔ slipRing:2
- Flush:24: slipRingMount_mainAxis:1 ↔ slipRing:2
- Mate:244: Insert M3 D5 L5mm:13 ↔ link_mainaxis_to_horArm:1
- Flush:25: Insert M3 D5 L5mm:13 ↔ link_mainaxis_to_horArm:1
- Mate:245: Insert M3 D5 L5mm:13 ↔ DIN EN ISO 4027 M3 x 16:1
- Mate:246: Insert M3 D5 L5mm_MIR2:1 ↔ DIN EN ISO 4027 M3 x 16:2
- Mate:247: Insert M3 D5 L5mm_MIR2:1 ↔ link_mainaxis_to_horArm:1
- Flush:26: Insert M3 D5 L5mm_MIR2:1 ↔ link_mainaxis_to_horArm:1
- Flush:27 (-2 mm): DIN EN ISO 4027 M3 x 16:2 ↔ link_mainaxis_to_horArm:1
- Flush:28 (-2 mm): DIN EN ISO 4027 M3 x 16:1 ↔ link_mainaxis_to_horArm:1
- Mate:248: sensormout_pendulum:1 ↔ DIN EN ISO 4762 M3 x 8:2
- Mate:249: pendulum_1:1 ↔ Insert M3 D5 L5mm_MIR1:1
- Flush:29: pendulum_1:1 ↔ Insert M3 D5 L5mm_MIR1:1
